# Autodesk Inventor assembly: Assembly1
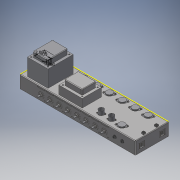
[picture p0: Inventor's stored thumbnail of the model, 180x180]
Saved by Autodesk Inventor 2016 (Build 200138000, 138)
## iProperties
Created: 2015-10-14
Part Number: Assembly1
Document SubType Name: Assembly
Designer: jeremyhale
Author: jeremyhale
## Documents named in this file (31)
- \\psf\Home\Documents\Poorhouse\git\p0001\chassis.iam
- chassis.iam
- \\psf\Home\Documents\Poorhouse\git\p0001\chassis.ipt
- \\psf\Home\Documents\Poorhouse\git\p0001\tube socket 8 pin.ipt
- \\psf\Home\Documents\Poorhouse\git\p0001\tube socket 9 pin.ipt
- \\psf\Home\Documents\Poorhouse\git\p0001\xmfr power.ipt
- \\psf\Home\Documents\Poorhouse\git\p0001\xmfr output.ipt
- \\psf\Home\Documents\Inventor\Content Center Files\R2016\en-US\AS 1427(08)\AS 1427 - M3 x 5(6) I.ipt
- \\psf\Home\Documents\Inventor\Content Center Files\R2016\en-US\AS 1474(1)\AS 1474 - M2.5(1).ipt
- \\psf\Home\Documents\Inventor\Content Center Files\R2016\en-US\AS 1474(1)\AS 1474 - M3.5(1).ipt
- \\psf\Home\Documents\Inventor\Content Center Files\R2016\en-US\AS 1474(1)\AS 1474 - M3(1).ipt
- \\psf\Home\Documents\Poorhouse\git\p0001\iec320_703W-00_04.ipt
- \\psf\Home\Documents\Inventor\Content Center Files\R2016\en-US\AS 1427(07)\AS 1427 - M3 x 10(6) II.ipt
- \\psf\Home\Documents\Poorhouse\git\p0001\Toggle Large A.ipt
- \\psf\Home\Documents\Poorhouse\git\p0001\AUDIO JACK 2.ipt
- \\psf\Home\Documents\Poorhouse\git\p0001\12ax7_complete.ipt
- \\psf\Home\Documents\Poorhouse\git\p0001\Noval socket.ipt
- \\psf\Home\Documents\Poorhouse\git\p0001\octal assembly.ipt
- \\psf\Home\Documents\Poorhouse\git\p0001\el34 assembly_r1.ipt
- \\psf\Home\Documents\Poorhouse\git\p0001\Bussman fuse holder HKP - 0,25'' X 1,25''.ipt
- \\psf\Home\Documents\Poorhouse\git\p0001\cage nut m6.iam
- \\psf\Home\Documents\Poorhouse\git\p0001\PEC11R-4220F-S0024.ipt
- \\psf\Home\Documents\Inventor\Content Center Files\R2016\en-US\UNI 5590  A\UNI 5590 - A M7.ipt
- \\psf\Home\Documents\Inventor\Content Center Files\R2016\en-US\BS 4320(2)\BS 4320 - M7 (Form B).ipt
- \\psf\Home\Documents\Poorhouse\git\p0001\rotary control.iam
- \\psf\Home\Documents\Poorhouse\git\p0001\Standoff 7mm M2 Wurth 9774070243R.ipt
- \\psf\Home\Documents\Poorhouse\git\p0001\chassis\Design Accelerator\Bolted Connection2.iam
- \\psf\Home\Documents\Poorhouse\git\p0001\chassis\Design Accelerator\Bolted Connection3.iam
- \\psf\Home\Documents\Poorhouse\git\p0001\chassis\Design Accelerator\Bolted Connection4.iam
- \\psf\Home\Documents\Poorhouse\git\p0001\chassis\Design Accelerator\Bolted Connection5.iam
- \\psf\Home\Documents\Poorhouse\git\p0001\chassis\Design Accelerator\Bolted Connection8.iam
## Components (214 placed, 28 different names)
1. chassis:1 — Rotational:1, Rotational:2, Rotational:3, Rotational:4, Rotational:5, Rotational:6, Rotational:7, Rotational:8, Rotational:9, Rotational:10, Mate:4, Insert:20, Insert:21, Insert:22, Insert:23, Insert:24, Insert:25, Insert:26, Insert:27, Insert:28, Insert:29, Insert:30, Insert:31, Insert:32, Insert:33, Insert:34, Insert:35, Insert:36, Insert:37, Rotational:11, Rotational:12, Mate:11, Mate:13, Rigid:15, Rigid:18, Rigid:19, Rigid:20, Rotational:15, Rotational:16, Rotational:17, Rotational:18, Rotational:19, Rotational:20, Rigid:22, Rigid:23, Flush:1, Flush:2, Flush:3, Rigid:24, Rigid:25, Rigid:26, Mate:16, Mate:19, Mate:20, Mate:29, Mate:31, Mate:33, Rotational:27, Rotational:28, Mate:37
2. big preamp tube sockets — Rotational:3, Rotational:4, Insert:13, Insert:14
3. xmfr power:1 — Rotational:7, Rotational:8
4. xmfr output:1 — Rotational:9, Rotational:10
5. Bussman fuse holder HKP - 0,25'' X 1,25'':1 — Rigid:22
6. PowerSwitch — Rigid:23
7. AS 1474 - Metric M2.5:1 — Mate:3, Mate:4
8. AS 1474 - Metric M3.5:1 — Insert:20
9. AS 1474 - Metric M3.5:2 — Insert:21
10. AS 1474 - Metric M3.5:3 — Insert:22
11. AS 1474 - Metric M3.5:4 — Insert:23
12. AS 1474 - Metric M3.5:5 — Insert:24
13. AS 1474 - Metric M3.5:6 — Insert:25
14. AS 1474 - Metric M3.5:7 — Insert:26
15. AS 1474 - Metric M3.5:8 — Insert:27
16. AS 1474 - Metric M3.5:9 — Insert:28
17. AS 1474 - Metric M3.5:10 — Insert:29
18. AS 1474 - Metric M3.5:11 — Insert:30
19. AS 1474 - Metric M3.5:12 — Insert:31
20. AS 1474 - Metric M3.5:13 — Insert:32
21. AS 1474 - Metric M3.5:14 — Insert:33
22. AS 1474 - Metric M3:1 — Insert:34
23. AS 1474 - Metric M3:2 — Insert:35
24. AS 1474 - Metric M3:3 — Insert:36
25. AS 1474 - Metric M3:4 — Insert:37
26. AS 1427 Z - Metric M3 x 5:1 — Insert:1, Mate:3
27. AS 1427 Z - Metric M3 x 5:2 — Insert:2
28. AS 1427 Z - Metric M3 x 5:3 — Insert:3
29. AS 1427 Z - Metric M3 x 5:4 — Insert:4
30. AS 1427 Z - Metric M3 x 5:5 — Insert:5
31. AS 1427 Z - Metric M3 x 5:6 — Insert:6
32. AS 1427 Z - Metric M3 x 5:7 — Insert:7
33. AS 1427 Z - Metric M3 x 5:8 — Insert:8
34. AS 1427 Z - Metric M3 x 5:9 — Insert:9
35. AS 1427 Z - Metric M3 x 5:10 — Insert:10
36. AS 1427 Z - Metric M3 x 5:11 — Insert:11
37. AS 1427 Z - Metric M3 x 5:12 — Insert:12
38. AS 1427 Z - Metric M3 x 5:13 — Insert:13
39. AS 1427 Z - Metric M3 x 5:14 — Insert:14
40. AS 1427 Z - Metric M3 x 5:15 — Insert:15
41. AS 1427 Z - Metric M3 x 5:16 — Insert:16
42. AS 1427 Z - Metric M3 x 5:17 — Insert:17
43. AS 1427 Z - Metric M3 x 5:18 — Insert:18
44. iec320_703W-00_04:1 — Rotational:11, Rotational:12, Mate:6, Mate:7
45. AS 1427 Z - Metric M3 x 10:2 — Mate:6, Mate:10
46. AS 1427 Z - Metric M3 x 10:1 — Mate:7, Mate:12
47. AS 1474 - Metric M3:5 — Mate:10, Mate:11
48. AS 1474 - Metric M3:6 — Mate:12, Mate:13
49. 12ax7_complete:1 — Rotational:13
50. 12ax7_complete:2 — Rotational:14
51. Noval socket:1 — Rigid:18, Rotational:13
52. Noval socket:2 — Rigid:19, Rotational:14
53. octal assembly:1 — Rigid:20
54. octal assembly:2 — Rotational:15, Rotational:21
55. octal assembly:3 — Rotational:16, Rotational:22
56. octal assembly:4 — Rotational:18, Rotational:23
57. octal assembly:5 — Rotational:17, Rigid:21
58. octal assembly:6 — Rotational:19, Rotational:24
59. octal assembly:7 — Rotational:20, Rotational:25
60. el34 assembly_r1:1 — Rotational:21
61. el34 assembly_r1:2 — Rotational:22
62. el34 assembly_r1:3 — Rigid:21
63. el34 assembly_r1:4 — Rotational:23
64. el34 assembly_r1:5 — Rotational:24
65. el34 assembly_r1:6 — Rotational:25
66. tube socket 8 pin:1 — Rotational:1, Rotational:2, Insert:1, Insert:2
67. tube socket 8 pin:2 — Insert:3, Insert:4
68. tube socket 8 pin:3 — Insert:5, Insert:6
69. tube socket 8 pin:4 — Insert:7, Insert:8
70. tube socket 8 pin:5 — Insert:15, Insert:16
71. tube socket 8 pin:6 — Insert:17, Insert:18
72. tube socket 9 pin:1 — Rotational:5, Rotational:6, Insert:9, Insert:10
73. tube socket 9 pin:2 — Insert:11, Insert:12
74. Speaker — Rigid:15
75. AUDIO JACK 2:3
76. AUDIO JACK 2:4
77. cage nut m6:1 [sub-assembly] — Rigid:24
78. cage nut m6:2 [sub-assembly]
79. cage nut m6:3 [sub-assembly]
80. cage nut m6:4 [sub-assembly]
81. cage nut m6:5 [sub-assembly] — Rigid:25
82. cage nut m6:6 [sub-assembly]
83. cage nut m6:7 [sub-assembly] — Rigid:26
84. cage nut m6:8 [sub-assembly]
85. Input Jack — Rotational:27
86. AUDIO JACK 2:5
87. Bolted Connection:4 [sub-assembly] — Mate:37, Mate:38
88. Bolted Connection:3 [sub-assembly] — Mate:29, Mate:30
89. Bolted Connection:2 [sub-assembly] — Mate:31, Mate:32
90. Bolted Connection:1 [sub-assembly] — Mate:33, Mate:34
91. Standoff 7mm M2 Wurth 9774070243R:4 — Insert:42, Mate:20, Mate:38
92. Standoff 7mm M2 Wurth 9774070243R:3 — Insert:41, Mate:32
93. Standoff 7mm M2 Wurth 9774070243R:2 — Insert:40, Mate:30
94. Standoff 7mm M2 Wurth 9774070243R:1 — Insert:39, Mate:19, Mate:34
95. rotary control:1 [sub-assembly] — Insert:39, Insert:40, Insert:41, Insert:42, Rotational:26, Angle:1, Cylindrical:1, Mate:39, Mate:40
96. BS 4320 Form AB M7 (Form B):1 — Mate:15, Mate:16, Mate:18
97. UNI 5590 A A M7:1 — Mate:17, Mate:18
98. PEC11R-4220F-S0024:1 — Mate:15, Mate:17, Rotational:26, Cylindrical:1, Rotational:28
99. Bolted Connection:37 [sub-assembly]
100. Bolted Connection:38 [sub-assembly]
101. Bolted Connection:39 [sub-assembly]
102. Bolted Connection:40 [sub-assembly]
103. Standoff 7mm M2 Wurth 9774070243R:5
104. Standoff 7mm M2 Wurth 9774070243R:6
105. Standoff 7mm M2 Wurth 9774070243R:7
106. Standoff 7mm M2 Wurth 9774070243R:8
107. rotary control:2 [sub-assembly]
108. BS 4320 Form AB M7 (Form B):2
109. UNI 5590 A A M7:2
110. PEC11R-4220F-S0024:2
111. Bolted Connection:45 [sub-assembly]
112. Bolted Connection:46 [sub-assembly]
113. Bolted Connection:47 [sub-assembly]
114. Bolted Connection:48 [sub-assembly]
115. Standoff 7mm M2 Wurth 9774070243R:9
116. Standoff 7mm M2 Wurth 9774070243R:10
117. Standoff 7mm M2 Wurth 9774070243R:11
118. Standoff 7mm M2 Wurth 9774070243R:12
119. rotary control:3 [sub-assembly]
120. BS 4320 Form AB M7 (Form B):3
121. UNI 5590 A A M7:3
122. PEC11R-4220F-S0024:3
123. Bolted Connection:53 [sub-assembly]
124. Bolted Connection:54 [sub-assembly]
125. Bolted Connection:55 [sub-assembly]
126. Bolted Connection:56 [sub-assembly]
127. Standoff 7mm M2 Wurth 9774070243R:13
128. Standoff 7mm M2 Wurth 9774070243R:14
129. Standoff 7mm M2 Wurth 9774070243R:15
130. Standoff 7mm M2 Wurth 9774070243R:16
131. rotary control:4 [sub-assembly]
132. BS 4320 Form AB M7 (Form B):4
133. UNI 5590 A A M7:4
134. PEC11R-4220F-S0024:4
135. Bolted Connection:61 [sub-assembly]
136. Bolted Connection:62 [sub-assembly]
137. Bolted Connection:63 [sub-assembly]
138. Bolted Connection:64 [sub-assembly]
139. Standoff 7mm M2 Wurth 9774070243R:17
140. Standoff 7mm M2 Wurth 9774070243R:18
141. Standoff 7mm M2 Wurth 9774070243R:19
142. Standoff 7mm M2 Wurth 9774070243R:20
143. rotary control:5 [sub-assembly]
144. BS 4320 Form AB M7 (Form B):5
145. UNI 5590 A A M7:5
146. PEC11R-4220F-S0024:5
147. Bolted Connection:69 [sub-assembly]
148. Bolted Connection:70 [sub-assembly]
149. Bolted Connection:71 [sub-assembly]
150. Bolted Connection:72 [sub-assembly]
151. Standoff 7mm M2 Wurth 9774070243R:21
152. Standoff 7mm M2 Wurth 9774070243R:22
153. Standoff 7mm M2 Wurth 9774070243R:23
154. Standoff 7mm M2 Wurth 9774070243R:24
155. rotary control:6 [sub-assembly]
156. BS 4320 Form AB M7 (Form B):6
157. UNI 5590 A A M7:6
158. PEC11R-4220F-S0024:6
159. Bolted Connection:77 [sub-assembly]
160. Bolted Connection:78 [sub-assembly]
161. Bolted Connection:79 [sub-assembly]
162. Bolted Connection:80 [sub-assembly]
163. Standoff 7mm M2 Wurth 9774070243R:25
164. Standoff 7mm M2 Wurth 9774070243R:26
165. Standoff 7mm M2 Wurth 9774070243R:27
166. Standoff 7mm M2 Wurth 9774070243R:28
167. rotary control:7 [sub-assembly]
168. BS 4320 Form AB M7 (Form B):7
169. UNI 5590 A A M7:7
170. PEC11R-4220F-S0024:7
171. Bolted Connection:85 [sub-assembly]
172. Bolted Connection:86 [sub-assembly]
173. Bolted Connection:87 [sub-assembly]
174. Bolted Connection:88 [sub-assembly]
175. Standoff 7mm M2 Wurth 9774070243R:29
176. Standoff 7mm M2 Wurth 9774070243R:30
177. Standoff 7mm M2 Wurth 9774070243R:31
178. Standoff 7mm M2 Wurth 9774070243R:32
179. rotary control:8 [sub-assembly]
180. BS 4320 Form AB M7 (Form B):8
181. UNI 5590 A A M7:8
182. PEC11R-4220F-S0024:8
183. Bolted Connection:33 [sub-assembly] — Mate:39, Mate:40
184. Bolted Connection:34 [sub-assembly]
185. Bolted Connection:35 [sub-assembly]
186. Bolted Connection:36 [sub-assembly]
187. Bolted Connection:41 [sub-assembly]
188. Bolted Connection:42 [sub-assembly]
189. Bolted Connection:43 [sub-assembly]
190. Bolted Connection:44 [sub-assembly]
191. Bolted Connection:49 [sub-assembly]
192. Bolted Connection:50 [sub-assembly]
193. Bolted Connection:51 [sub-assembly]
194. Bolted Connection:52 [sub-assembly]
195. Bolted Connection:57 [sub-assembly]
196. Bolted Connection:58 [sub-assembly]
197. Bolted Connection:59 [sub-assembly]
198. Bolted Connection:60 [sub-assembly]
199. Bolted Connection:65 [sub-assembly]
200. Bolted Connection:66 [sub-assembly]
201. Bolted Connection:67 [sub-assembly]
202. Bolted Connection:68 [sub-assembly]
203. Bolted Connection:73 [sub-assembly]
204. Bolted Connection:74 [sub-assembly]
205. Bolted Connection:75 [sub-assembly]
206. Bolted Connection:76 [sub-assembly]
207. Bolted Connection:81 [sub-assembly]
208. Bolted Connection:82 [sub-assembly]
209. Bolted Connection:83 [sub-assembly]
210. Bolted Connection:84 [sub-assembly]
211. Bolted Connection:89 [sub-assembly]
212. Bolted Connection:90 [sub-assembly]
213. Bolted Connection:91 [sub-assembly]
214. Bolted Connection:92 [sub-assembly]
## Component patterns: Big Tube Sockets (6 elements), small preamp tube sockets (2 elements), speaker jacks (3 elements), Cage Nuts Top (4 elements), Cage Nuts Right (2 elements), Cage Nuts Left (2 elements), input jacks (2 elements), controls (8 elements), (4 elements, first: Bolted Connection:33), Component Pattern 21:2 (4 elements), Component Pattern 21:3 (4 elements), Component Pattern 21:4 (4 elements), Component Pattern 21:5 (4 elements), Component Pattern 21:6 (4 elements), Component Pattern 21:7 (4 elements), Component Pattern 21:8 (4 elements)
## Relationships (107: Insert 40, RevoluteJoint 28, Mate 24, WeldJoint 10, Flush 3, Angle 1, CylindricalJoint 1)
- Rotational:1 [RevoluteJoint]: chassis:1 ↔ tube socket 8 pin:1
- Rotational:2 [RevoluteJoint]: chassis:1 ↔ tube socket 8 pin:1
- Rotational:3 [RevoluteJoint]: chassis:1 ↔ big preamp tube sockets
- Rotational:4 [RevoluteJoint]: chassis:1 ↔ big preamp tube sockets
- Rotational:5 [RevoluteJoint]: chassis:1 ↔ tube socket 9 pin:1
- Rotational:6 [RevoluteJoint]: chassis:1 ↔ tube socket 9 pin:1
- Rotational:7 [RevoluteJoint]: chassis:1 ↔ xmfr power:1
- Rotational:8 [RevoluteJoint]: chassis:1 ↔ xmfr power:1
- Rotational:9 [RevoluteJoint]: chassis:1 ↔ xmfr output:1
- Rotational:10 [RevoluteJoint]: chassis:1 ↔ xmfr output:1
- Insert:1: AS 1427 Z - Metric M3 x 5:1 ↔ tube socket 8 pin:1
- Insert:2: AS 1427 Z - Metric M3 x 5:2 ↔ tube socket 8 pin:1
- Insert:3: AS 1427 Z - Metric M3 x 5:3 ↔ tube socket 8 pin:2
- Insert:4: AS 1427 Z - Metric M3 x 5:4 ↔ tube socket 8 pin:2
- Insert:5: AS 1427 Z - Metric M3 x 5:5 ↔ tube socket 8 pin:3
- Insert:6: AS 1427 Z - Metric M3 x 5:6 ↔ tube socket 8 pin:3
- Insert:7: AS 1427 Z - Metric M3 x 5:7 ↔ tube socket 8 pin:4
- Insert:8: AS 1427 Z - Metric M3 x 5:8 ↔ tube socket 8 pin:4
- Insert:9: AS 1427 Z - Metric M3 x 5:9 ↔ tube socket 9 pin:1
- Insert:10: AS 1427 Z - Metric M3 x 5:10 ↔ tube socket 9 pin:1
- Insert:11: AS 1427 Z - Metric M3 x 5:11 ↔ tube socket 9 pin:2
- Insert:12: AS 1427 Z - Metric M3 x 5:12 ↔ tube socket 9 pin:2
- Insert:13: big preamp tube sockets ↔ AS 1427 Z - Metric M3 x 5:13
- Insert:14: big preamp tube sockets ↔ AS 1427 Z - Metric M3 x 5:14
- Insert:15: AS 1427 Z - Metric M3 x 5:15 ↔ tube socket 8 pin:5
- Insert:16: AS 1427 Z - Metric M3 x 5:16 ↔ tube socket 8 pin:5
- Insert:17: AS 1427 Z - Metric M3 x 5:17 ↔ tube socket 8 pin:6
- Insert:18: AS 1427 Z - Metric M3 x 5:18 ↔ tube socket 8 pin:6
- Mate:3: AS 1474 - Metric M2.5:1 ↔ AS 1427 Z - Metric M3 x 5:1
- Mate:4: chassis:1 ↔ AS 1474 - Metric M2.5:1
- Insert:20: chassis:1 ↔ AS 1474 - Metric M3.5:1
- Insert:21: chassis:1 ↔ AS 1474 - Metric M3.5:2
- Insert:22: chassis:1 ↔ AS 1474 - Metric M3.5:3
- Insert:23: chassis:1 ↔ AS 1474 - Metric M3.5:4
- Insert:24: chassis:1 ↔ AS 1474 - Metric M3.5:5
- Insert:25: chassis:1 ↔ AS 1474 - Metric M3.5:6
- Insert:26: chassis:1 ↔ AS 1474 - Metric M3.5:7
- Insert:27: chassis:1 ↔ AS 1474 - Metric M3.5:8
- Insert:28: chassis:1 ↔ AS 1474 - Metric M3.5:9
- Insert:29: chassis:1 ↔ AS 1474 - Metric M3.5:10
- Insert:30: chassis:1 ↔ AS 1474 - Metric M3.5:11
- Insert:31: chassis:1 ↔ AS 1474 - Metric M3.5:12
- Insert:32: chassis:1 ↔ AS 1474 - Metric M3.5:13
- Insert:33: chassis:1 ↔ AS 1474 - Metric M3.5:14
- Insert:34: chassis:1 ↔ AS 1474 - Metric M3:1
- Insert:35: chassis:1 ↔ AS 1474 - Metric M3:2
- Insert:36: chassis:1 ↔ AS 1474 - Metric M3:3
- Insert:37: chassis:1 ↔ AS 1474 - Metric M3:4
- Rotational:11 [RevoluteJoint]: chassis:1 ↔ iec320_703W-00_04:1
- Rotational:12 [RevoluteJoint]: chassis:1 ↔ iec320_703W-00_04:1
- Mate:6: iec320_703W-00_04:1 ↔ AS 1427 Z - Metric M3 x 10:2
- Mate:7: iec320_703W-00_04:1 ↔ AS 1427 Z - Metric M3 x 10:1
- Mate:10: AS 1427 Z - Metric M3 x 10:2 ↔ AS 1474 - Metric M3:5
- Mate:11: chassis:1 ↔ AS 1474 - Metric M3:5
- Mate:12: AS 1427 Z - Metric M3 x 10:1 ↔ AS 1474 - Metric M3:6
- Mate:13: chassis:1 ↔ AS 1474 - Metric M3:6
- Rigid:15 [WeldJoint]: chassis:1 ↔ Speaker
- Rigid:18 [WeldJoint]: chassis:1 ↔ Noval socket:1
- Rigid:19 [WeldJoint]: chassis:1 ↔ Noval socket:2
- Rotational:13 [RevoluteJoint]: 12ax7_complete:1 ↔ Noval socket:1
- Rotational:14 [RevoluteJoint]: 12ax7_complete:2 ↔ Noval socket:2
- Rigid:20 [WeldJoint]: chassis:1 ↔ octal assembly:1
- Rotational:15 [RevoluteJoint]: chassis:1 ↔ octal assembly:2
- Rotational:16 [RevoluteJoint]: chassis:1 ↔ octal assembly:3
- Rotational:17 [RevoluteJoint]: chassis:1 ↔ octal assembly:5
- Rotational:18 [RevoluteJoint]: chassis:1 ↔ octal assembly:4
- Rotational:19 [RevoluteJoint]: chassis:1 ↔ octal assembly:6
- Rotational:20 [RevoluteJoint]: chassis:1 ↔ octal assembly:7
- Rotational:21 [RevoluteJoint]: octal assembly:2 ↔ el34 assembly_r1:1
- Rotational:22 [RevoluteJoint]: octal assembly:3 ↔ el34 assembly_r1:2
- Rigid:21 [WeldJoint]: octal assembly:5 ↔ el34 assembly_r1:3
- Rotational:23 [RevoluteJoint]: octal assembly:4 ↔ el34 assembly_r1:4
- Rotational:24 [RevoluteJoint]: octal assembly:6 ↔ el34 assembly_r1:5
- Rotational:25 [RevoluteJoint]: octal assembly:7 ↔ el34 assembly_r1:6
- Rigid:22 [WeldJoint]: chassis:1 ↔ Bussman fuse holder HKP - 0,25'' X 1,25'':1
- Rigid:23 [WeldJoint]: chassis:1 ↔ PowerSwitch
- Flush:1: chassis:1
- Flush:2: chassis:1
- Flush:3: chassis:1
- Rigid:24 [WeldJoint]: chassis:1 ↔ cage nut m6:1
- Rigid:25 [WeldJoint]: chassis:1 ↔ cage nut m6:5
- Rigid:26 [WeldJoint]: chassis:1 ↔ cage nut m6:7
- Mate:15: BS 4320 Form AB M7 (Form B):1 ↔ PEC11R-4220F-S0024:1
- Mate:16: chassis:1 ↔ BS 4320 Form AB M7 (Form B):1
- Mate:17: UNI 5590 A A M7:1 ↔ PEC11R-4220F-S0024:1
- Mate:18: BS 4320 Form AB M7 (Form B):1 ↔ UNI 5590 A A M7:1
- Insert:39: Standoff 7mm M2 Wurth 9774070243R:1 ↔ rotary control:1
- Insert:40: Standoff 7mm M2 Wurth 9774070243R:2 ↔ rotary control:1
- Insert:41: Standoff 7mm M2 Wurth 9774070243R:3 ↔ rotary control:1
- Insert:42: Standoff 7mm M2 Wurth 9774070243R:4 ↔ rotary control:1
- Mate:19: chassis:1 ↔ Standoff 7mm M2 Wurth 9774070243R:1
- Mate:20: chassis:1 ↔ Standoff 7mm M2 Wurth 9774070243R:4
- Rotational:26 [RevoluteJoint]: rotary control:1 ↔ PEC11R-4220F-S0024:1
- Angle:1 (0 deg): rotary control:1
- Cylindrical:1: rotary control:1 ↔ PEC11R-4220F-S0024:1
- Mate:29: chassis:1 ↔ Bolted Connection:3
- Mate:30: Bolted Connection:3 ↔ Standoff 7mm M2 Wurth 9774070243R:2
- Mate:31: chassis:1 ↔ Bolted Connection:2
- Mate:32: Bolted Connection:2 ↔ Standoff 7mm M2 Wurth 9774070243R:3
- Mate:33: chassis:1 ↔ Bolted Connection:1
- Mate:34: Bolted Connection:1 ↔ Standoff 7mm M2 Wurth 9774070243R:1
- Rotational:27 [RevoluteJoint]: chassis:1 ↔ Input Jack
- Rotational:28 [RevoluteJoint]: chassis:1 ↔ PEC11R-4220F-S0024:1
- Mate:37: chassis:1 ↔ Bolted Connection:4
- Mate:38: Bolted Connection:4 ↔ Standoff 7mm M2 Wurth 9774070243R:4
- Mate:39: rotary control:1 ↔ Bolted Connection:33
- Mate:40: rotary control:1 ↔ Bolted Connection:33
## Named parameters: ControlSpacing = 44.45 mm
